# Autodesk Inventor assembly: Шкаф 1дв
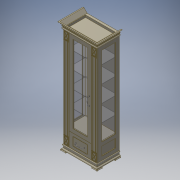
[picture p0: Inventor's stored thumbnail of the model, 180x180]
Saved by Autodesk Inventor 2019 (Build 230136000, 136)
## iProperties
Created: 2018-09-22
Part Number: Шкаф 1дв
Material: Типовые
Document SubType Name: Assembly
Designer: Андреев Н.Л.
Mass: 66597.7 g
Surface Area: 118811 cm^2
Volume: 74367.6 cm^3
Density: 0.895521 g/cm^3
Author: Андреев Н.Л.
## Documents named in this file (21)
- C:\Users\andrnl\Documents\Inventor\Мурзин\Шкаф 1дв.iam
- C:\Users\andrnl\Documents\Inventor\Мурзин\Ш1Д Стенка боковая.ipt
- C:\Users\andrnl\Documents\Inventor\Мурзин\Ш1Д Стенка задняя.ipt
- C:\Users\andrnl\Documents\Inventor\Мурзин\Ш1Д Пилястра.ipt
- C:\Users\andrnl\Documents\Inventor\Мурзин\Ш1Д Фасад ящика.ipt
- C:\Users\andrnl\Documents\Inventor\Мурзин\Ш1Д Дверца.ipt
- C:\Users\andrnl\Documents\Inventor\Мурзин\Ш1Д Дно.ipt
- C:\Users\andrnl\Documents\Inventor\Мурзин\Ш1Д Цоколь.ipt
- C:\Users\andrnl\Documents\Inventor\Мурзин\Ш1Д Ножка.ipt
- C:\Users\andrnl\Documents\Inventor\Мурзин\Ш1Д Планка цоколя.ipt
- C:\Users\andrnl\Documents\Inventor\Мурзин\Ш1Д Филенка бок.ipt
- C:\Users\andrnl\Documents\Inventor\Мурзин\Ш1Д Стекло бок.ipt
- C:\Users\andrnl\Documents\Inventor\Мурзин\Ш1Д Стекло дверцы.ipt
- C:\Users\andrnl\Documents\Inventor\Мурзин\Ш1Д Полка.ipt
- C:\Users\andrnl\Documents\Inventor\Мурзин\Ш1Д Потолок.ipt
- C:\Users\andrnl\Documents\Inventor\Мурзин\Ш1Д Цоколь верха.ipt
- C:\Users\andrnl\Documents\Inventor\Мурзин\Ш1Д Планка верха.ipt
- C:\Users\andrnl\Documents\Inventor\Мурзин\Ш1Д Карниз.ipt
- C:\Users\andrnl\Documents\Inventor\Мурзин\Ш1Д Шашечки.ipt
- C:\Users\andrnl\Documents\Inventor\Мурзин\Ш1Д Полка стекло.ipt
- C:\Users\andrnl\Documents\Inventor\Мурзин\Ручка скоба.ipt
## Components (31 placed, 20 different names)
1. Ш1Д Стенка боковая:1
2. Ш1Д Стенка задняя:1
3. Ш1Д Пилястра:1
4. Ш1Д Фасад ящика:1 — Совмещение:9, Совмещение:10, Совмещение:11
5. Ш1Д Дверца:1 — Совмещение:6, Совмещение:7
6. Ш1Д Дно:1
7. Ш1Д Цоколь:1 — Касательность:1
8. Ш1Д Ножка:1 — Совмещение:5
9. Ш1Д Планка цоколя:1
10. Ш1Д Филенка бок:1
11. Ш1Д Полка:1
12. Ш1Д Потолок:1
13. Ш1Д Цоколь верха:1
14. Ш1Д Планка верха:1
15. Ш1Д Карниз:1
16. Ш1Д Шашечки:1
17. Ш1Д Стенка боковая:2
18. Ш1Д Пилястра:2
19. Ш1Д Филенка бок:2
20. Ш1Д Ножка:2 — Совмещение:2
21. Ш1Д Ножка:3 — Совмещение:3, Совмещение:4, Совмещение:5
22. Ш1Д Ножка:4 — Совмещение:1, Совмещение:2, Касательность:1, Совмещение:4
23. Ш1Д Стекло бок:1
24. Ш1Д Стекло дверцы:1
25. Ш1Д Стекло бок:2
26. Ручка скоба:1 — Совмещение:6, Совмещение:7, Совмещение:8
27. Ручка скоба:2 — Совмещение:9, Совмещение:10, Совмещение:11
28. Ш1Д Полка стекло:1
29. Ш1Д Полка стекло:2
30. Ш1Д Полка стекло:3
31. Ш1Д Полка стекло:4
## Component patterns: (4 elements, first: Ш1Д Полка стекло:1)
## Relationships (12: Mate 11, Tangent 1)
- Совмещение:1 [Mate]: Ш1Д Ножка:4
- Совмещение:2 [Mate]: Ш1Д Ножка:2 ↔ Ш1Д Ножка:4
- Касательность:1 [Tangent]: Ш1Д Цоколь:1 ↔ Ш1Д Ножка:4
- Совмещение:3 [Mate]: Ш1Д Ножка:3
- Совмещение:4 [Mate]: Ш1Д Ножка:3 ↔ Ш1Д Ножка:4
- Совмещение:5 [Mate]: Ш1Д Ножка:1 ↔ Ш1Д Ножка:3
- Совмещение:6 [Mate]: Ш1Д Дверца:1 ↔ Ручка скоба:1
- Совмещение:7 [Mate] (-35 mm): Ш1Д Дверца:1 ↔ Ручка скоба:1
- Совмещение:8 [Mate] (1000 mm): Ручка скоба:1
- Совмещение:9 [Mate]: Ш1Д Фасад ящика:1 ↔ Ручка скоба:2
- Совмещение:10 [Mate]: Ш1Д Фасад ящика:1 ↔ Ручка скоба:2
- Совмещение:11 [Mate]: Ш1Д Фасад ящика:1 ↔ Ручка скоба:2
